# Autodesk Inventor assembly: lenkung
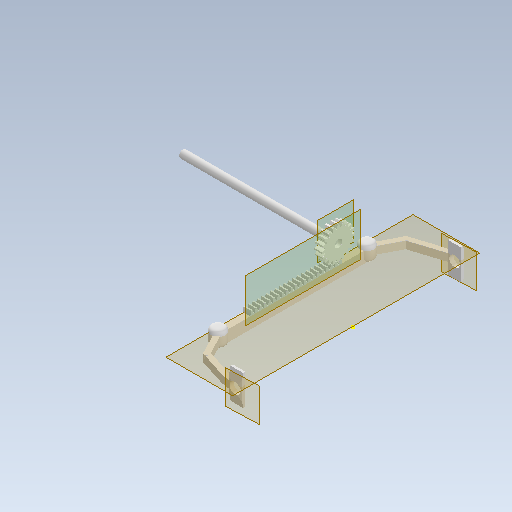
[picture p0: Inventor's stored thumbnail of the model, 512x512]
Saved by Autodesk Inventor 2021 (Build 250183000, 183)
## iProperties
Created: 2021-01-15
Part Number: lenkung
Document SubType Name: Assembly
Designer: LETPJG
Author: LETPJG
## Documents named in this file (5)
- C:\Users\LETPJG\Documents\Inventor\zahnstange\lenkung.iam
- C:\Users\LETPJG\Documents\Inventor\zahnstange\Bauteil15.ipt
- C:\Users\LETPJG\Documents\Inventor\zahnstange\Bauteil16.ipt
- C:\Users\LETPJG\Documents\Inventor\zahnstange\Zahnstange.iam
- C:\Users\LETPJG\Documents\Inventor\zahnstange\Bauteil1.ipt
## Components (4 placed, 4 different names)
1. Bauteil15:1 — Passend:2, Passend:3, Fluchtend:1, Passend:4
2. Zahnstange:1 [sub-assembly] — Passend:2, Passend:3, Fluchtend:1, Fluchtend:2, Passend:5
3. Bauteil16:1 — Passend:4
4. Bauteil1:1 — Passend:5
## Relationships (6: Mate 4, Flush 2)
- Passend:2 [Mate]: Bauteil15:1 ↔ Zahnstange:1
- Passend:3 [Mate]: Bauteil15:1 ↔ Zahnstange:1
- Fluchtend:1 [Flush]: Bauteil15:1 ↔ Zahnstange:1
- Passend:4 [Mate]: Bauteil15:1 ↔ Bauteil16:1
- Fluchtend:2 [Flush]: Zahnstange:1
- Passend:5 [Mate]: Zahnstange:1 ↔ Bauteil1:1
